# Autodesk Inventor assembly: Assembly3
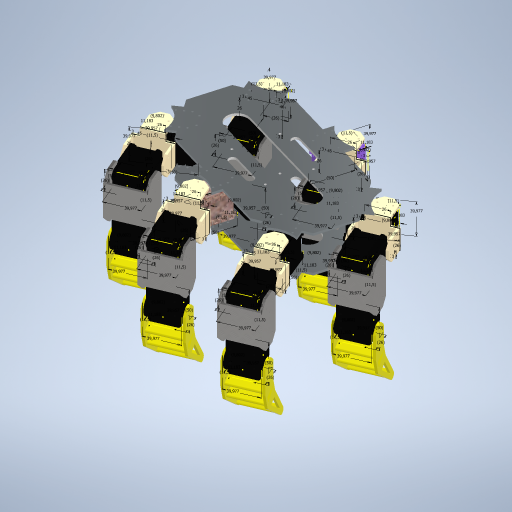
[picture p0: Inventor's stored thumbnail of the model, 512x512]
Saved by Autodesk Inventor 2024 (Build 280153000, 153)
## iProperties
Created: 2024-02-16
Part Number: Assembly3
Document SubType Name: Assembly
Designer: kamil
Author: kamil
## Documents named in this file (6)
- D:\Projects\Robotics\Hexapod\Assembly3.iam
- D:\Projects\Robotics\Hexapod\first_junction.ipt
- D:\Projects\Robotics\Hexapod\AX-12A\AX-12A.iam
- D:\Projects\Robotics\Hexapod\second_junction.ipt
- D:\Projects\Robotics\Hexapod\leg_part.ipt
- D:\Projects\Robotics\Hexapod\base.ipt
## Components (38 placed, 5 different names)
1. first_junction:1 — Mate:1, Mate:2, Mate:3, Mate:4, Mate:5, Mate:6, Mate:7
2. AX-12A:1 [sub-assembly] — Mate:1, Mate:2, Mate:3, Mate:4, Mate:103, Mate:104, Mate:105
3. AX-12A:2 [sub-assembly] — Mate:5, Mate:6, Mate:7, Mate:14, Mate:18, Mate:19
4. second_junction:1 — Mate:11, Mate:12, Mate:13, Mate:14, Mate:18, Mate:19
5. AX-12A:3 [sub-assembly] — Mate:11, Mate:12, Mate:13, Mate:15, Mate:16, Mate:17
6. leg_part:1 — Mate:15, Mate:16, Mate:17
7. first_junction:2 — Mate:120
8. AX-12A:4 [sub-assembly] — Mate:100, Mate:101, Mate:102, Mate:118, Mate:119
9. AX-12A:5 [sub-assembly]
10. second_junction:2
11. AX-12A:6 [sub-assembly]
12. leg_part:2
13. first_junction:3
14. AX-12A:7 [sub-assembly] — Mate:106, Mate:107, Mate:108
15. AX-12A:8 [sub-assembly]
16. second_junction:3
17. AX-12A:9 [sub-assembly]
18. leg_part:3
19. first_junction:4
20. AX-12A:10 [sub-assembly] — Mate:109, Mate:110, Mate:111
21. AX-12A:11 [sub-assembly]
22. second_junction:4
23. AX-12A:12 [sub-assembly]
24. leg_part:4
25. first_junction:5
26. AX-12A:13 [sub-assembly] — Mate:115, Mate:116, Mate:117
27. AX-12A:14 [sub-assembly]
28. second_junction:5
29. AX-12A:15 [sub-assembly]
30. leg_part:5
31. first_junction:6
32. AX-12A:16 [sub-assembly] — Mate:112, Mate:113, Mate:114
33. AX-12A:17 [sub-assembly]
34. second_junction:6
35. AX-12A:18 [sub-assembly]
36. leg_part:6
37. base:1 — Mate:100, Mate:101, Mate:102, Mate:103, Mate:104, Mate:105, Mate:106, Mate:107, Mate:108, Mate:109, Mate:110, Mate:111, Mate:112, Mate:113, Mate:114, Mate:115, Mate:116, Mate:117
38. base:2 — Mate:118, Mate:119, Mate:120
## Relationships (117: Mate 117)
- Mate:1: first_junction:1 ↔ AX-12A:1
- Mate:2: first_junction:1 ↔ AX-12A:1
- Mate:3: first_junction:1 ↔ AX-12A:1
- Mate:4: first_junction:1 ↔ AX-12A:1
- Mate:5: first_junction:1 ↔ AX-12A:2
- Mate:6: first_junction:1 ↔ AX-12A:2
- Mate:7: first_junction:1 ↔ AX-12A:2
- Mate:11: second_junction:1 ↔ AX-12A:3
- Mate:12: second_junction:1 ↔ AX-12A:3
- Mate:13: second_junction:1 ↔ AX-12A:3
- Mate:14: AX-12A:2 ↔ second_junction:1
- Mate:15: AX-12A:3 ↔ leg_part:1
- Mate:16: AX-12A:3 ↔ leg_part:1
- Mate:17: AX-12A:3 ↔ leg_part:1
- Mate:18: AX-12A:2 ↔ second_junction:1
- Mate:19: AX-12A:2 ↔ second_junction:1
- [Mate]: first_junction:2 ↔ AX-12A:4
- [Mate]: first_junction:2 ↔ AX-12A:4
- [Mate]: first_junction:2 ↔ AX-12A:4
- [Mate]: first_junction:2 ↔ AX-12A:4
- [Mate]: first_junction:2 ↔ AX-12A:5
- [Mate]: first_junction:2 ↔ AX-12A:5
- [Mate]: first_junction:2 ↔ AX-12A:5
- [Mate]: second_junction:2 ↔ AX-12A:6
- [Mate]: second_junction:2 ↔ AX-12A:6
- [Mate]: second_junction:2 ↔ AX-12A:6
- [Mate]: AX-12A:5 ↔ second_junction:2
- [Mate]: AX-12A:6 ↔ leg_part:2
- [Mate]: AX-12A:6 ↔ leg_part:2
- [Mate]: AX-12A:6 ↔ leg_part:2
- [Mate]: AX-12A:5 ↔ second_junction:2
- [Mate]: AX-12A:5 ↔ second_junction:2
- [Mate]: first_junction:3 ↔ AX-12A:7
- [Mate]: first_junction:3 ↔ AX-12A:7
- [Mate]: first_junction:3 ↔ AX-12A:7
- [Mate]: first_junction:3 ↔ AX-12A:7
- [Mate]: first_junction:3 ↔ AX-12A:8
- [Mate]: first_junction:3 ↔ AX-12A:8
- [Mate]: first_junction:3 ↔ AX-12A:8
- [Mate]: second_junction:3 ↔ AX-12A:9
- [Mate]: second_junction:3 ↔ AX-12A:9
- [Mate]: second_junction:3 ↔ AX-12A:9
- [Mate]: AX-12A:8 ↔ second_junction:3
- [Mate]: AX-12A:9 ↔ leg_part:3
- [Mate]: AX-12A:9 ↔ leg_part:3
- [Mate]: AX-12A:9 ↔ leg_part:3
- [Mate]: AX-12A:8 ↔ second_junction:3
- [Mate]: AX-12A:8 ↔ second_junction:3
- [Mate]: first_junction:4 ↔ AX-12A:10
- [Mate]: first_junction:4 ↔ AX-12A:10
- [Mate]: first_junction:4 ↔ AX-12A:10
- [Mate]: first_junction:4 ↔ AX-12A:10
- [Mate]: first_junction:4 ↔ AX-12A:11
- [Mate]: first_junction:4 ↔ AX-12A:11
- [Mate]: first_junction:4 ↔ AX-12A:11
- [Mate]: second_junction:4 ↔ AX-12A:12
- [Mate]: second_junction:4 ↔ AX-12A:12
- [Mate]: second_junction:4 ↔ AX-12A:12
- [Mate]: AX-12A:11 ↔ second_junction:4
- [Mate]: AX-12A:12 ↔ leg_part:4
- [Mate]: AX-12A:12 ↔ leg_part:4
- [Mate]: AX-12A:12 ↔ leg_part:4
- [Mate]: AX-12A:11 ↔ second_junction:4
- [Mate]: AX-12A:11 ↔ second_junction:4
- [Mate]: first_junction:5 ↔ AX-12A:13
- [Mate]: first_junction:5 ↔ AX-12A:13
- [Mate]: first_junction:5 ↔ AX-12A:13
- [Mate]: first_junction:5 ↔ AX-12A:13
- [Mate]: first_junction:5 ↔ AX-12A:14
- [Mate]: first_junction:5 ↔ AX-12A:14
- [Mate]: first_junction:5 ↔ AX-12A:14
- [Mate]: second_junction:5 ↔ AX-12A:15
- [Mate]: second_junction:5 ↔ AX-12A:15
- [Mate]: second_junction:5 ↔ AX-12A:15
- [Mate]: AX-12A:14 ↔ second_junction:5
- [Mate]: AX-12A:15 ↔ leg_part:5
- [Mate]: AX-12A:15 ↔ leg_part:5
- [Mate]: AX-12A:15 ↔ leg_part:5
- [Mate]: AX-12A:14 ↔ second_junction:5
- [Mate]: AX-12A:14 ↔ second_junction:5
- [Mate]: first_junction:6 ↔ AX-12A:16
- [Mate]: first_junction:6 ↔ AX-12A:16
- [Mate]: first_junction:6 ↔ AX-12A:16
- [Mate]: first_junction:6 ↔ AX-12A:16
- [Mate]: first_junction:6 ↔ AX-12A:17
- [Mate]: first_junction:6 ↔ AX-12A:17
- [Mate]: first_junction:6 ↔ AX-12A:17
- [Mate]: second_junction:6 ↔ AX-12A:18
- [Mate]: second_junction:6 ↔ AX-12A:18
- [Mate]: second_junction:6 ↔ AX-12A:18
- [Mate]: AX-12A:17 ↔ second_junction:6
- [Mate]: AX-12A:18 ↔ leg_part:6
- [Mate]: AX-12A:18 ↔ leg_part:6
- [Mate]: AX-12A:18 ↔ leg_part:6
- [Mate]: AX-12A:17 ↔ second_junction:6
- [Mate]: AX-12A:17 ↔ second_junction:6
- Mate:100: AX-12A:4 ↔ base:1
- Mate:101: AX-12A:4 ↔ base:1
- Mate:102: AX-12A:4 ↔ base:1
- Mate:103: AX-12A:1 ↔ base:1
- Mate:104: AX-12A:1 ↔ base:1
- Mate:105: AX-12A:1 ↔ base:1
- Mate:106: AX-12A:7 ↔ base:1
- Mate:107: AX-12A:7 ↔ base:1
- Mate:108: AX-12A:7 ↔ base:1
- Mate:109: AX-12A:10 ↔ base:1
- Mate:110: AX-12A:10 ↔ base:1
- Mate:111: AX-12A:10 ↔ base:1
- Mate:112: AX-12A:16 ↔ base:1
- Mate:113: AX-12A:16 ↔ base:1
- Mate:114: AX-12A:16 ↔ base:1
- Mate:115: AX-12A:13 ↔ base:1
- Mate:116: AX-12A:13 ↔ base:1
- Mate:117: AX-12A:13 ↔ base:1
- Mate:118: AX-12A:4 ↔ base:2
- Mate:119: AX-12A:4 ↔ base:2
- Mate:120: first_junction:2 ↔ base:2
## Named parameters: d99_d5 = 0 mm, d100_d6 = 0 mm, d101_d10 = 0 mm, d102_d11 = 0 mm, d103_d12 = 0 mm, d104_d13 = 0 mm, d105_d14 = 0 mm, d106_d15 = 0 mm, d107_d16 = 0 mm, d108_d17 = 0 mm, d109_d18 = 0 mm, d110_d0 = 0 mm, d111_d1 = 0 mm, d112_d2 = 0 mm, d113_d3 = 0 mm, d114_d4 = 0 mm, d115_d5 = 0 mm, d116_d6 = 0 mm, d117_d10 = 0 mm, d118_d11 = 0 mm, d119_d12 = 0 mm, d120_d13 = 0 mm, d121_d14 = 0 mm, d122_d15 = 0 mm, d123_d16 = 0 mm, d124_d17 = 0 mm, d125_d18 = 0 mm, d126_d0 = 0 mm, d127_d1 = 0 mm, d128_d2 = 0 mm, d129_d3 = 0 mm, d130_d4 = 0 mm, d131_d5 = 0 mm, d132_d6 = 0 mm, d133_d10 = 0 mm, d134_d11 = 0 mm, d135_d12 = 0 mm, d136_d13 = 0 mm, d137_d14 = 0 mm, d138_d15 = 0 mm, d139_d16 = 0 mm, d140_d17 = 0 mm, d141_d18 = 0 mm, d142_d0 = 0 mm, d143_d1 = 0 mm, d144_d2 = 0 mm, d145_d3 = 0 mm, d146_d4 = 0 mm, d147_d5 = 0 mm, d148_d6 = 0 mm, d149_d10 = 0 mm, d150_d11 = 0 mm, d151_d12 = 0 mm, d152_d13 = 0 mm, d153_d14 = 0 mm, d154_d15 = 0 mm, d155_d16 = 0 mm, d156_d17 = 0 mm, d157_d18 = 0 mm, d158_d0 = 0 mm, d159_d1 = 0 mm, d160_d2 = 0 mm, d161_d3 = 0 mm, d162_d4 = 0 mm, d163_d5 = 0 mm, d164_d6 = 0 mm, d165_d10 = 0 mm, d166_d11 = 0 mm, d167_d12 = 0 mm, d168_d13 = 0 mm, d169_d14 = 0 mm, d170_d15 = 0 mm, d171_d16 = 0 mm, d172_d17 = 0 mm, d173_d18 = 0 mm, d174_d0 = 0 mm, d175_d1 = 0 mm, d176_d2 = 0 mm, d177_d3 = 0 mm, d178_d4 = 0 mm
